# Autodesk Inventor assembly: capstone assembly
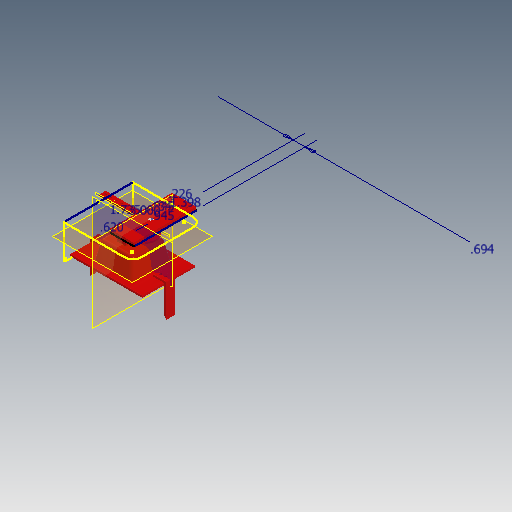
[picture p0: Inventor's stored thumbnail of the model, 512x512]
Saved by Autodesk Inventor 2020 (Build 240168000, 168)
## iProperties
Created: 2020-02-10
Part Number: capstone assembly
Document SubType Name: Assembly
Designer: ball
Author: ball
## Documents named in this file (7)
- C:\FTC\FTC8863CAD\2019 Robot\Delivery\Capstone\capstone assembly.iam
- C:\FTC\FTC8863CAD\2019 Robot\Delivery\Capstone\8863 capstone.3.ipt
- C:\FTC\FTC8863CAD\2019 Robot\Delivery\Capstone\capstone ear.ipt
- C:\FTC\FTC8863CAD\2019 Robot\Delivery\Capstone\capstone hook constant radius.ipt
- C:\FTC\FTC8863CAD\2019 Robot\Delivery\Capstone\capstone hook mount.ipt
- C:\FTC\FTC8863CAD\StepLibraries\Screws\M3 x 12 HEX HEAD CAP SCREW.ipt
- C:\FTC\FTC8863CAD\StepLibraries\Nuts\m3 18-8 STAINLESS STL NYLON-INSERT LOCKNUT.ipt
## Components (7 placed, 6 different names)
1. 8863 capstone.3:1 — Mate:1, Mate:2, Mate:3, Mate:4, Mate:5, Mate:6, Flush:2, Mate:11
2. capstone ear:1 — Mate:4, Mate:5, Mate:6
3. capstone ear:2 — Mate:1, Mate:2, Mate:3
4. capstone hook mount:1 — Flush:2, Rotational:2, Mate:10, Mate:12, Mate:13
5. capstone hook constant radius:1 — Rotational:2, Mate:10, Mate:11, Mate:14
6. M3 x 12 HEX HEAD CAP SCREW:1 — Mate:12, Mate:13, Mate:15
7. m3 18-8 STAINLESS STL NYLON-INSERT LOCKNUT:1 — Mate:14, Mate:15
## Relationships (14: Mate 12, Flush 1, RevoluteJoint 1)
- Mate:1: 8863 capstone.3:1 ↔ capstone ear:2
- Mate:2: 8863 capstone.3:1 ↔ capstone ear:2
- Mate:3: 8863 capstone.3:1 ↔ capstone ear:2
- Mate:4: 8863 capstone.3:1 ↔ capstone ear:1
- Mate:5: 8863 capstone.3:1 ↔ capstone ear:1
- Mate:6: 8863 capstone.3:1 ↔ capstone ear:1
- Flush:2: 8863 capstone.3:1 ↔ capstone hook mount:1
- Rotational:2 [RevoluteJoint]: capstone hook mount:1 ↔ capstone hook constant radius:1
- Mate:10: capstone hook mount:1 ↔ capstone hook constant radius:1
- Mate:11: 8863 capstone.3:1 ↔ capstone hook constant radius:1
- Mate:12: capstone hook mount:1 ↔ M3 x 12 HEX HEAD CAP SCREW:1
- Mate:13: capstone hook mount:1 ↔ M3 x 12 HEX HEAD CAP SCREW:1
- Mate:14: capstone hook constant radius:1 ↔ m3 18-8 STAINLESS STL NYLON-INSERT LOCKNUT:1
- Mate:15: M3 x 12 HEX HEAD CAP SCREW:1 ↔ m3 18-8 STAINLESS STL NYLON-INSERT LOCKNUT:1
